# Autodesk Inventor assembly: Servo and Frame
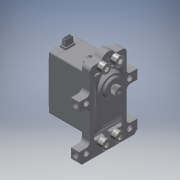
[picture p0: Inventor's stored thumbnail of the model, 180x180]
Saved by Autodesk Inventor 2019 (Build 230136000, 136)
## iProperties
Created: 2018-11-18
Part Number: Servo and Frame
Document SubType Name: Assembly
Designer: Ashley
Author: Ashley
## Documents named in this file (7)
- C:\Users\Ashley\Desktop\repositories\design\inventor\Imported Components\goBilda\Servo and Frame.iam
- C:\Users\Ashley\Desktop\repositories\design\inventor\Imported Components\goBilda\goBildaServo.ipt
- C:\Users\Ashley\Desktop\repositories\design\inventor\Imported Components\goBilda\1802SeriesServoFrame.ipt
- C:\Users\Ashley\Desktop\repositories\design\inventor\Imported Components\goBilda\Servo and Frame\Design Accelerator\Bolted Connection1.iam
- C:\Users\Ashley\Desktop\repositories\design\inventor\Imported Components\goBilda\Servo and Frame\Design Accelerator\Bolted Connection2.iam
- C:\Users\Ashley\Desktop\repositories\design\inventor\Imported Components\goBilda\Servo and Frame\Design Accelerator\Bolted Connection3.iam
- C:\Users\Ashley\Desktop\repositories\design\inventor\Imported Components\goBilda\Servo and Frame\Design Accelerator\Bolted Connection4.iam
## Components (6 placed, 3 different names)
1. goBildaServo:1 — Mate:1
2. 1802SeriesServoFrame:1 — Mate:1, Mate:2, Mate:3, Mate:4, Mate:5, Mate:6, Mate:7, Mate:8, Mate:9
3. Bolted Connection:1 [sub-assembly] — Mate:2, Mate:3
4. Bolted Connection:2 [sub-assembly] — Mate:4, Mate:5
5. Bolted Connection:3 [sub-assembly] — Mate:6, Mate:7
6. Bolted Connection:4 [sub-assembly] — Mate:8, Mate:9
## Relationships (9: Mate 9)
- Mate:1: goBildaServo:1 ↔ 1802SeriesServoFrame:1
- Mate:2: 1802SeriesServoFrame:1 ↔ Bolted Connection:1
- Mate:3: 1802SeriesServoFrame:1 ↔ Bolted Connection:1
- Mate:4: 1802SeriesServoFrame:1 ↔ Bolted Connection:2
- Mate:5: 1802SeriesServoFrame:1 ↔ Bolted Connection:2
- Mate:6: 1802SeriesServoFrame:1 ↔ Bolted Connection:3
- Mate:7: 1802SeriesServoFrame:1 ↔ Bolted Connection:3
- Mate:8: 1802SeriesServoFrame:1 ↔ Bolted Connection:4
- Mate:9: 1802SeriesServoFrame:1 ↔ Bolted Connection:4
